# Autodesk Inventor assembly: Assembly2
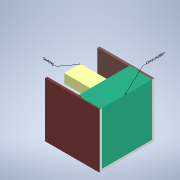
[picture p0: Inventor's stored thumbnail of the model, 180x180]
Saved by Autodesk Inventor 2022.3 (Build 263350000, 350)
## iProperties
Created: 2023-02-06
Part Number: Assembly2
Document SubType Name: Assembly
Designer: lbmcgill42
Author: lbmcgill42
## Documents named in this file (10)
- \\labdrive.tntech.edu\labdrive\lbmcgill42\Documents\Assembly2.iam
- \\labdrive.tntech.edu\labdrive\lbmcgill42\Documents\power_supply.ipt
- \\labdrive.tntech.edu\labdrive\lbmcgill42\Documents\Chips.ipt
- \\labdrive.tntech.edu\labdrive\lbmcgill42\Documents\Pedestal.ipt
- \\labdrive.tntech.edu\labdrive\lbmcgill42\Documents\Intake.ipt
- \\labdrive.tntech.edu\labdrive\lbmcgill42\Documents\Sorting.ipt
- \\labdrive.tntech.edu\labdrive\lbmcgill42\Documents\Jetson.ipt
- \\labdrive.tntech.edu\labdrive\lbmcgill42\Documents\Aduino.ipt
- \\labdrive.tntech.edu\labdrive\lbmcgill42\Documents\Arduino2.ipt
- \\labdrive.tntech.edu\labdrive\lbmcgill42\Documents\chassisFloor.ipt
## Components (9 placed, 9 different names)
1. power_supply:1 — Rigid:4
2. Chips:1 — Rigid:2
3. Pedestal:1 — Rigid:3
4. Intake:1 — Rigid:1
5. Sorting:1 — Rigid:8
6. Jetson:1 — Rigid:7
7. Aduino1:1 — Rigid:5
8. Arduino2:1 — Rigid:6
9. chassisFloor:1 — Rigid:1, Rigid:2, Rigid:3, Rigid:4, Rigid:5, Rigid:6, Rigid:7, Rigid:8
## Relationships (8: WeldJoint 8)
- Rigid:1 [WeldJoint]: Intake:1 ↔ chassisFloor:1
- Rigid:2 [WeldJoint]: Chips:1 ↔ chassisFloor:1
- Rigid:3 [WeldJoint]: Pedestal:1 ↔ chassisFloor:1
- Rigid:4 [WeldJoint]: power_supply:1 ↔ chassisFloor:1
- Rigid:5 [WeldJoint]: Aduino1:1 ↔ chassisFloor:1
- Rigid:6 [WeldJoint]: Arduino2:1 ↔ chassisFloor:1
- Rigid:7 [WeldJoint]: Jetson:1 ↔ chassisFloor:1
- Rigid:8 [WeldJoint]: Sorting:1 ↔ chassisFloor:1
